# Autodesk Inventor assembly: assembled servo block
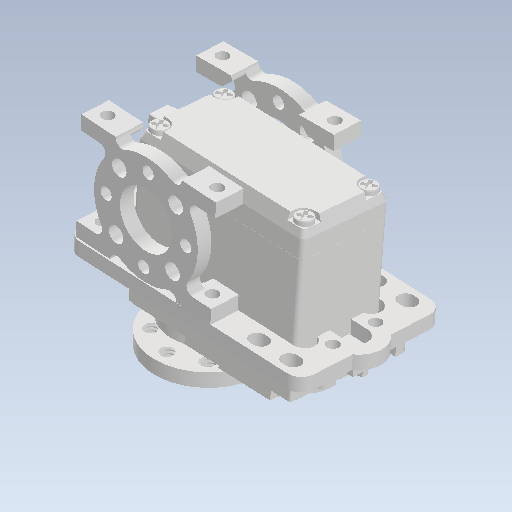
[picture p0: Inventor's stored thumbnail of the model, 512x512]
Saved by Autodesk Inventor 2020.1 (Build 241239000, 239)
## iProperties
Created: 2020-09-23
Part Number: assembled servo block
Document SubType Name: Assembly
Designer: elois
Author: elois
## Documents named in this file (5)
- C:\Users\elois\Documents\GitHub\CAD-2021-Ultimate_Goal\Wobble Goal\assembled servo block.iam
- C:\Users\elois\Documents\GitHub\CAD-2021-Ultimate_Goal\ServoCity\servo mount.ipt
- C:\Users\elois\Documents\GitHub\CAD-2021-Ultimate_Goal\ServoCity\servo side brackets.ipt
- C:\Users\elois\Documents\GitHub\CAD-2021-Ultimate_Goal\ServoCity\go builda servo(speed).ipt
- C:\Users\elois\Documents\GitHub\CAD-2021-Ultimate_Goal\ServoCity\525125_MIR.ipt
## Components (5 placed, 4 different names)
1. servo mount:1 — Mate:1, Mate:2, Mate:3, Mate:21, Mate:22, Mate:23
2. servo side brackets:1 — Mate:23
3. go builda servo(speed):1 — Mate:1, Mate:2, Mate:3, Mate:21, Mate:24
4. 525125_MIR:1 — Mate:24
5. servo side brackets:2 — Mate:22
## Relationships (7: Mate 7)
- Mate:1: servo mount:1 ↔ go builda servo(speed):1
- Mate:2: servo mount:1 ↔ go builda servo(speed):1
- Mate:3: servo mount:1 ↔ go builda servo(speed):1
- Mate:21: servo mount:1 ↔ go builda servo(speed):1
- Mate:22: servo mount:1 ↔ servo side brackets:2
- Mate:23: servo mount:1 ↔ servo side brackets:1
- Mate:24: go builda servo(speed):1 ↔ 525125_MIR:1
